# Autodesk Inventor assembly: Countdown Clock Assembly
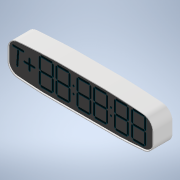
[picture p0: Inventor's stored thumbnail of the model, 180x180]
Saved by Autodesk Inventor 2021 (Build 250183000, 183)
## iProperties
Created: 2020-06-27
Part Number: Countdown Clock Assembly
Document SubType Name: Assembly
Designer: dech3
Author: dech3
## Documents named in this file (5)
- D:\Inventor\CountDown Clock Project\Countdown Clock Assembly.iam
- D:\Inventor\CountDown Clock Project\7 Segment Clock Face.ipt
- D:\Inventor\CountDown Clock Project\7 Segment Clock Blanking Plate.ipt
- D:\Inventor\CountDown Clock Project\7 Segment Clock Shell.ipt
- D:\Inventor\CountDown Clock Project\LED Clock Lights.ipt
## Components (5 placed, 5 different names)
1. 7 Segment Clock Face:1 — Mate:1
2. 7 Segment Clock Blanking Plate:1 — Mate:1
3. 7 Segment Clock Blanking Plate:Black
4. 7 Segment Clock Shell:1
5. LED Clock Lights:1
## Relationships (1: Mate 1)
- Mate:1: 7 Segment Clock Face:1 ↔ 7 Segment Clock Blanking Plate:1
